# Autodesk Inventor assembly: PWTR-0157
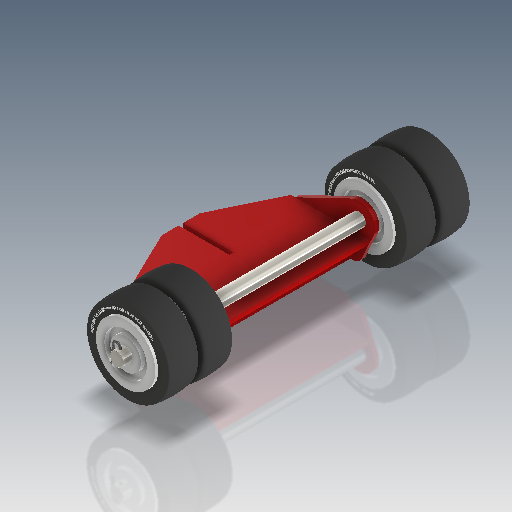
[picture p0: Inventor's stored thumbnail of the model, 512x512]
Saved by Autodesk Inventor 2021.1 (Build 251245000, 245)
## iProperties
Created: 2020-09-03
Part Number: PWTR-0157
Document SubType Name: Assembly
Designer: alid
Author: alid
## Documents named in this file (6)
- C:\Vault Workspace\Design Data\Projects\PRJ0095\PWTR-CTO\PWTR-0157.iam
- C:\Vault Workspace\Design Data\Projects\PRJ0095\PWTR-CTO\PWTR-0135.ipt
- C:\Vault Workspace\Design Data\Projects\PRJ0095\PWTR-CTO\PWTR-0138.ipt
- C:\Vault Workspace\Design Data\Projects\PRJ0095\PWTR-CTO\PWTR-0139.ipt
- C:\Vault Workspace\Design Data\Projects\PRJ0095\PWTR-CTO\PWTR-0114.ipt
- C:\Vault Workspace\Design Data\Projects\PRJ0095\PWTR-CTO\PWTR-0158.ipt
## Components (8 placed, 6 different names)
1. Wheel Bracket — Insert:1, Insert:2, Insert:3, Insert:4
2. PWTR-0158:1 — Insert:1, Rigid:1
3. PWTR-0138:1 — Insert:2
4. Wheel — Insert:3, Insert:6
5. PWTR-0139:2 — Insert:4, Insert:5
6. PWTR-0114:1 — Rigid:1
7. PWTR-0139:3 — Insert:5
8. PWTR-0139:4 — Insert:6
## Relationships (7: Insert 6, WeldJoint 1)
- Insert:1 (80 mm): Wheel Bracket ↔ PWTR-0158:1
- Insert:2 (40 mm): Wheel Bracket ↔ PWTR-0138:1
- Insert:3: Wheel Bracket ↔ Wheel
- Insert:4: Wheel Bracket ↔ PWTR-0139:2
- Rigid:1 [WeldJoint]: PWTR-0158:1 ↔ PWTR-0114:1
- Insert:5: PWTR-0139:2 ↔ PWTR-0139:3
- Insert:6: Wheel ↔ PWTR-0139:4
